# Autodesk Inventor assembly: platform
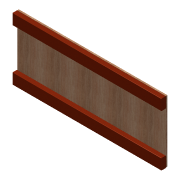
[picture p0: Inventor's stored thumbnail of the model, 180x180]
Saved by Autodesk Inventor 2015 (Build 190159000, 159)
## iProperties
Created: 2015-01-03
Part Number: platform
Document SubType Name: Assembly
Designer: Peter
Author: Peter
## Documents named in this file (3)
- T:\FILES\Inventor 2015 Projects\ScoringPlatform\platform.iam
- T:\FILES\Inventor 2015 Projects\ScoringPlatform\plywood platform.ipt
- T:\FILES\Inventor 2015 Projects\ScoringPlatform\2x4x48.ipt
## Components (3 placed, 2 different names)
1. plywood platform:1 — Mate:1, Flush:1, Flush:2, Rigid:1
2. 2x4x48:1 — Mate:1, Flush:1, Flush:2
3. 2x4x48:2 — Rigid:1
## Relationships (4: Flush 2, Mate 1, WeldJoint 1)
- Mate:1: plywood platform:1 ↔ 2x4x48:1
- Flush:1: plywood platform:1 ↔ 2x4x48:1
- Flush:2: plywood platform:1 ↔ 2x4x48:1
- Rigid:1 [WeldJoint]: plywood platform:1 ↔ 2x4x48:2
